# Autodesk Inventor assembly: WoodenSocket
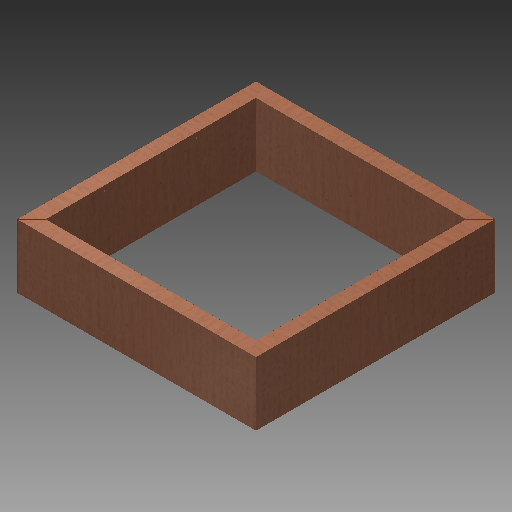
[picture p0: Inventor's stored thumbnail of the model, 512x512]
Saved by Autodesk Inventor 2019.3 (Build 233278000, 278)
## iProperties
Created: 2019-01-12
Part Number: WoodenSocket
Material: Generisch
Document SubType Name: Assembly
Designer: Jonas
Author: Jonas
## Documents named in this file (4)
- C:\Users\Jonas\Desktop\RGBCube\RGBCubev2\CAD\Socket\WoodenSocket.iam
- C:\Users\Jonas\Desktop\RGBCube\RGBCubev2\CAD\Socket\Front.ipt
- C:\Users\Jonas\Desktop\RGBCube\RGBCubev2\CAD\Socket\Back.ipt
- C:\Users\Jonas\Desktop\RGBCube\RGBCubev2\CAD\Socket\Side.ipt
## Components (4 placed, 4 different names)
1. Front:1 — Passend:1, Passend:6, Passend:11, Passend:13, Passend:14
2. Back:1 — Passend:7, Passend:9, Passend:12
3. Side:Right — Passend:8, Passend:9, Passend:13, Passend:18
4. Side:Left — Passend:10, Passend:11, Passend:12, Passend:15, Passend:16, Passend:17
## Relationships (14: Mate 14)
- Passend:1 [Mate]: Front:1
- Passend:6 [Mate]: Front:1
- Passend:7 [Mate]: Back:1
- Passend:8 [Mate]: Side:Right
- Passend:9 [Mate]: Back:1 ↔ Side:Right
- Passend:10 [Mate]: Side:Left
- Passend:11 [Mate]: Front:1 ↔ Side:Left
- Passend:12 [Mate]: Back:1 ↔ Side:Left
- Passend:13 [Mate]: Front:1 ↔ Side:Right
- Passend:14 [Mate]: Front:1
- Passend:15 [Mate]: Side:Left
- Passend:16 [Mate]: Side:Left
- Passend:17 [Mate]: Side:Left
- Passend:18 [Mate]: Side:Right
